# Autodesk Inventor assembly: 1130_Watery Rotary Union Assembly_V1
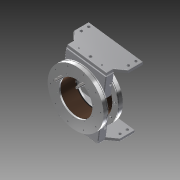
[picture p0: Inventor's stored thumbnail of the model, 180x180]
Saved by Autodesk Inventor 2020 (Build 240168000, 168)
## iProperties
Created: 2019-03-26
Part Number: 1130_Watery Rotary Union Assembly_V1
Document SubType Name: Assembly
Designer: e22ma
Author: e22ma
## Documents named in this file (11)
- C:\Users\RFLab\Dropbox\MPI Group Folder\fMPI (Rodent)\Small Bore Imager_Open Source Files\Inventor Files\1xxx_Rotating Gantry\11xx_Magnet Assembly\1130_Watery Rotary Union Assembly_V1.iam
- C:\Users\RFLab\Dropbox\MPI Group Folder\fMPI (Rodent)\Small Bore Imager_Open Source Files\Inventor Files\1xxx_Rotating Gantry\11xx_Magnet Assembly\113x_Water Rotary Union Assembly\1136_RU Top Plate_V1.ipt
- C:\Users\RFLab\Dropbox\MPI Group Folder\fMPI (Rodent)\Small Bore Imager_Open Source Files\Inventor Files\1xxx_Rotating Gantry\11xx_Magnet Assembly\113x_Water Rotary Union Assembly\1137_RU Mechanical Connector_V1.ipt
- C:\Users\RFLab\Dropbox\MPI Group Folder\fMPI (Rodent)\Small Bore Imager_Open Source Files\Inventor Files\1xxx_Rotating Gantry\11xx_Magnet Assembly\113x_Water Rotary Union Assembly\1131_Inner RU Body_V1.ipt
- C:\Users\RFLab\Dropbox\MPI Group Folder\fMPI (Rodent)\Small Bore Imager_Open Source Files\Inventor Files\1xxx_Rotating Gantry\11xx_Magnet Assembly\113x_Water Rotary Union Assembly\1132_Outer RU Body_V1.ipt
- C:\Users\RFLab\Dropbox\MPI Group Folder\fMPI (Rodent)\Small Bore Imager_Open Source Files\Inventor Files\1xxx_Rotating Gantry\11xx_Magnet Assembly\113x_Water Rotary Union Assembly\1133_RU End Cap.ipt
- C:\Users\RFLab\Dropbox\MPI Group Folder\fMPI (Rodent)\Small Bore Imager_Open Source Files\Inventor Files\1xxx_Rotating Gantry\11xx_Magnet Assembly\113x_Water Rotary Union Assembly\1134_RU O Ring Cap_V1.ipt
- C:\Users\RFLab\Dropbox\MPI Group Folder\fMPI (Rodent)\Small Bore Imager_Open Source Files\Inventor Files\1xxx_Rotating Gantry\11xx_Magnet Assembly\113x_Water Rotary Union Assembly\1138_Inner Gasket_V1.ipt
- C:\Users\RFLab\Dropbox\MPI Group Folder\fMPI (Rodent)\Small Bore Imager_Open Source Files\Inventor Files\1xxx_Rotating Gantry\11xx_Magnet Assembly\113x_Water Rotary Union Assembly\1135_Sq O Ring_V1.ipt
- C:\Users\RFLab\Dropbox\MPI Group Folder\fMPI (Rodent)\Small Bore Imager_Open Source Files\Inventor Files\1xxx_Rotating Gantry\11xx_Magnet Assembly\113x_Water Rotary Union Assembly\1139_Outer Gasket_V1.ipt
- C:\Users\RFLab\Dropbox\MPI Group Folder\fMPI (Rodent)\Small Bore Imager_Open Source Files\Inventor Files\1xxx_Rotating Gantry\11xx_Magnet Assembly\113x_Water Rotary Union Assembly\11310_Pipe Inserts_V1.ipt
## Components (18 placed, 10 different names)
1. 1131_Inner RU Body_V1:1 — Mate:1, Mate:2, Mate:3, Angle:1, Flush:1, Mate:20, Mate:21, Mate:24, Mate:25
2. 1132_Outer RU Body_V1:1 — Mate:1, Mate:2, Mate:5, Mate:6, Rotational:1, Mate:10, Mate:19, Angle:2, Mate:28
3. 1133_RU End Cap:1 — Flush:1, Flush:2, Flush:3, Mate:12, Flush:6, Flush:8, Flush:10, Mate:23
4. 1133_RU End Cap:2 — Mate:5, Rotational:1, Mate:13, Rigid:1, Rigid:2, Mate:15, Mate:16, Mate:17
5. 1134_RU O Ring Cap_V1:1 — Mate:6, Flush:4, Mate:13, Mate:18
6. 1137_RU Mechanical Connector_V1:1 — Flush:4, Mate:19, Flush:13, Mate:26, Angle:3, Flush:15, Flush:16
7. 1134_RU O Ring Cap_V1:2 — Mate:10, Mate:12, Mate:14
8. 1135_Sq O Ring_V1:1 — Flush:6
9. 1139_Outer Gasket_V1:1 — Flush:8, Mate:14
10. 1138_Inner Gasket_V1:1 — Flush:10
11. 1135_Sq O Ring_V1:2 — Rigid:2
12. 1139_Outer Gasket_V1:2 — Rigid:1, Mate:18
13. 1138_Inner Gasket_V1:2 — Mate:15, Mate:16, Mate:17
14. 11310_Pipe Inserts_V1:1 — Mate:20, Mate:21, Mate:23
15. 11310_Pipe Inserts_V1:2 — Mate:24, Mate:25
16. 1136_RU Top Plate_V1:1 — Flush:13, Mate:26, Angle:2, Angle:3
17. 1137_RU Mechanical Connector_V1:2 — Mate:28, Flush:15, Flush:16
18. 1136_RU Top Plate_V1:2
## Relationships (40: Mate 22, Flush 11, Angle 4, WeldJoint 2, RevoluteJoint 1)
- Mate:1: 1131_Inner RU Body_V1:1 ↔ 1132_Outer RU Body_V1:1
- Mate:2: 1131_Inner RU Body_V1:1 ↔ 1132_Outer RU Body_V1:1
- Mate:3: 1131_Inner RU Body_V1:1
- Angle:1 (0 deg): 1131_Inner RU Body_V1:1
- Flush:1: 1131_Inner RU Body_V1:1 ↔ 1133_RU End Cap:1
- Flush:2: 1133_RU End Cap:1
- Flush:3: 1133_RU End Cap:1
- Mate:5: 1132_Outer RU Body_V1:1 ↔ 1133_RU End Cap:2
- Mate:6: 1132_Outer RU Body_V1:1 ↔ 1134_RU O Ring Cap_V1:1
- Rotational:1 [RevoluteJoint]: 1132_Outer RU Body_V1:1 ↔ 1133_RU End Cap:2
- Flush:4: 1134_RU O Ring Cap_V1:1 ↔ 1137_RU Mechanical Connector_V1:1
- Mate:10: 1132_Outer RU Body_V1:1 ↔ 1134_RU O Ring Cap_V1:2
- Mate:12: 1133_RU End Cap:1 ↔ 1134_RU O Ring Cap_V1:2
- Mate:13: 1133_RU End Cap:2 ↔ 1134_RU O Ring Cap_V1:1
- Flush:6: 1133_RU End Cap:1 ↔ 1135_Sq O Ring_V1:1
- Flush:8: 1133_RU End Cap:1 ↔ 1139_Outer Gasket_V1:1
- Flush:10: 1133_RU End Cap:1 ↔ 1138_Inner Gasket_V1:1
- Mate:14: 1134_RU O Ring Cap_V1:2 ↔ 1139_Outer Gasket_V1:1
- Rigid:1 [WeldJoint]: 1133_RU End Cap:2 ↔ 1139_Outer Gasket_V1:2
- Rigid:2 [WeldJoint]: 1133_RU End Cap:2 ↔ 1135_Sq O Ring_V1:2
- Mate:15: 1133_RU End Cap:2 ↔ 1138_Inner Gasket_V1:2
- Mate:16: 1133_RU End Cap:2 ↔ 1138_Inner Gasket_V1:2
- Mate:17: 1133_RU End Cap:2 ↔ 1138_Inner Gasket_V1:2
- Mate:18: 1134_RU O Ring Cap_V1:1 ↔ 1139_Outer Gasket_V1:2
- Mate:19: 1132_Outer RU Body_V1:1 ↔ 1137_RU Mechanical Connector_V1:1
- Flush:13: 1137_RU Mechanical Connector_V1:1 ↔ 1136_RU Top Plate_V1:1
- Mate:20: 1131_Inner RU Body_V1:1 ↔ 11310_Pipe Inserts_V1:1
- Mate:21: 1131_Inner RU Body_V1:1 ↔ 11310_Pipe Inserts_V1:1
- Mate:23: 1133_RU End Cap:1 ↔ 11310_Pipe Inserts_V1:1
- Mate:24: 1131_Inner RU Body_V1:1 ↔ 11310_Pipe Inserts_V1:2
- Mate:25: 1131_Inner RU Body_V1:1 ↔ 11310_Pipe Inserts_V1:2
- Mate:26: 1137_RU Mechanical Connector_V1:1 ↔ 1136_RU Top Plate_V1:1
- Angle:2 (0 deg): 1132_Outer RU Body_V1:1 ↔ 1136_RU Top Plate_V1:1
- Angle:3 (0 deg): 1137_RU Mechanical Connector_V1:1 ↔ 1136_RU Top Plate_V1:1
- [Flush]: 1137_RU Mechanical Connector_V1:2 ↔ 1136_RU Top Plate_V1:2
- [Mate]: 1137_RU Mechanical Connector_V1:2 ↔ 1136_RU Top Plate_V1:2
- [Angle] (0 deg): 1137_RU Mechanical Connector_V1:2 ↔ 1136_RU Top Plate_V1:2
- Mate:28: 1132_Outer RU Body_V1:1 ↔ 1137_RU Mechanical Connector_V1:2
- Flush:15: 1137_RU Mechanical Connector_V1:1 ↔ 1137_RU Mechanical Connector_V1:2
- Flush:16: 1137_RU Mechanical Connector_V1:1 ↔ 1137_RU Mechanical Connector_V1:2
## Named parameters: d107_d104 = 0 mm, d108_d106 = 0 deg, d109_d84 = 0 mm
